# Autodesk Inventor assembly: asse_s_tstage
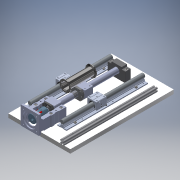
[picture p0: Inventor's stored thumbnail of the model, 180x180]
Saved by Autodesk Inventor 2019 (Build 230136000, 136)
## iProperties
Created: 2022-09-02
Part Number: asse_s_tstage
Document SubType Name: Assembly
Designer: kananovicha
Author: kananovicha
## Documents named in this file (10)
- C:\Users\kananovicha\Documents\work\workAppState\prj_shocksL\s_tstage\drawingsGit\s_tstage\asse_s_tstage\asse_s_tstage.iam
- C:\Users\kananovicha\Documents\work\workAppState\prj_shocksL\s_tstage\drawingsGit\s_tstage\mplate\mplate.ipt
- C:\Users\kananovicha\Documents\work\workAppState\prj_shocksL\s_tstage\drawingsGit\s_tstage\3rdParty\ballScrewAssembly\2510 L=400.iam
- C:\Users\kananovicha\Documents\work\workAppState\prj_shocksL\s_tstage\drawingsGit\s_tstage\allmainparams\allmainparams.ipt
- C:\Users\kananovicha\Documents\work\workAppState\prj_shocksL\s_tstage\drawingsGit\s_tstage\3rdParty\KF40nipple\qf40-150-n.iam
- C:\Users\kananovicha\Documents\work\workAppState\prj_shocksL\s_tstage\drawingsGit\s_tstage\3rdParty\br20-shaft-and-support-rail-resizable-1.snapshot.13\BR20\BR20-400.iam
- C:\Users\kananovicha\Documents\work\workAppState\prj_shocksL\s_tstage\drawingsGit\s_tstage\3rdParty\mod-sbr20uu-open-linear-bearing-1.snapshot.2\SBR20UU.iam
- C:\Users\kananovicha\Documents\work\workAppState\prj_shocksL\s_tstage\drawingsGit\s_tstage\tslot2020short\tslot2020short.ipt
- C:\Users\kananovicha\Documents\work\workAppState\prj_shocksL\s_tstage\drawingsGit\s_tstage\3rdParty\fasteners\ANSI B18.3.1M - M8x1.25 x 50(1).ipt
- C:\Users\kananovicha\Documents\work\workAppState\prj_shocksL\s_tstage\drawingsGit\s_tstage\3rdParty\fasteners\91290A328_Alloy Steel Socket Head Screw.ipt
## Components (26 placed, 8 different names)
1. mplate:1 — Flush:1, Mate:1, Mate:2, Mate:3, Mate:4, Angle:1, Angle:2, Angle:3, Flush:4, Mate:7, Flush:5, Flush:6
2. 2510 L=400:1 [sub-assembly] — Flush:1, Mate:1, Mate:2, Mate:5, Mate:6, Insert:1, Insert:2, Insert:3, Insert:4, Insert:5, Insert:6
3. qf40-150-n:1 [sub-assembly]
4. BR20-400:1 [sub-assembly] — Mate:3, Cylindrical:1, Angle:2, Mate:5, Mate:8, Flush:5, Insert:7
5. BR20-400:2 [sub-assembly] — Mate:4, Cylindrical:2, Mate:6, Flush:6, Insert:8
6. SBR20UU:1 [sub-assembly] — Cylindrical:1, Angle:1
7. SBR20UU:2 [sub-assembly] — Cylindrical:2, Angle:3
8. tslot2020short:1 — Flush:4, Mate:7, Mate:8
9. ANSI B18.3.1M - M8x1.25 x 50(1):1 — Insert:1
10. ANSI B18.3.1M - M8x1.25 x 50(1):2 — Insert:2
11. ANSI B18.3.1M - M8x1.25 x 50(1):3 — Insert:3
12. ANSI B18.3.1M - M8x1.25 x 50(1):4 — Insert:4
13. ANSI B18.3.1M - M8x1.25 x 50(1):5 — Insert:5
14. ANSI B18.3.1M - M8x1.25 x 50(1):6 — Insert:6
15. 91290A328_Alloy Steel Socket Head Screw:1 — Insert:7
16. 91290A328_Alloy Steel Socket Head Screw:3
17. 91290A328_Alloy Steel Socket Head Screw:4
18. 91290A328_Alloy Steel Socket Head Screw:5
19. 91290A328_Alloy Steel Socket Head Screw:6
20. 91290A328_Alloy Steel Socket Head Screw:7
21. 91290A328_Alloy Steel Socket Head Screw:2 — Insert:8
22. 91290A328_Alloy Steel Socket Head Screw:8
23. 91290A328_Alloy Steel Socket Head Screw:9
24. 91290A328_Alloy Steel Socket Head Screw:10
25. 91290A328_Alloy Steel Socket Head Screw:11
26. 91290A328_Alloy Steel Socket Head Screw:12
## Component patterns: (6 elements, first: 91290A328_Alloy Steel Socket Head Screw:1), (6 elements, first: 91290A328_Alloy Steel Socket Head Screw:2)
## Relationships (25: Mate 8, Insert 8, Flush 4, Angle 3, CylindricalJoint 2)
- Flush:1 (68.58 mm): mplate:1 ↔ 2510 L=400:1
- Mate:1: mplate:1 ↔ 2510 L=400:1
- Mate:2: mplate:1 ↔ 2510 L=400:1
- Mate:3: mplate:1 ↔ BR20-400:1
- Mate:4: mplate:1 ↔ BR20-400:2
- Cylindrical:1: BR20-400:1 ↔ SBR20UU:1
- Angle:1 (0 deg): mplate:1 ↔ SBR20UU:1
- Angle:2 (0 deg): mplate:1 ↔ BR20-400:1
- Cylindrical:2: BR20-400:2 ↔ SBR20UU:2
- Angle:3 (0 deg): mplate:1 ↔ SBR20UU:2
- Mate:5 (12.7 mm): 2510 L=400:1 ↔ BR20-400:1
- Mate:6 (12.7 mm): 2510 L=400:1 ↔ BR20-400:2
- Flush:4: mplate:1 ↔ tslot2020short:1
- Mate:7: mplate:1 ↔ tslot2020short:1
- Mate:8 (38.354 mm): BR20-400:1 ↔ tslot2020short:1
- Insert:1: 2510 L=400:1 ↔ ANSI B18.3.1M - M8x1.25 x 50(1):1
- Insert:2: 2510 L=400:1 ↔ ANSI B18.3.1M - M8x1.25 x 50(1):2
- Insert:3: 2510 L=400:1 ↔ ANSI B18.3.1M - M8x1.25 x 50(1):3
- Insert:4: 2510 L=400:1 ↔ ANSI B18.3.1M - M8x1.25 x 50(1):4
- Insert:5: 2510 L=400:1 ↔ ANSI B18.3.1M - M8x1.25 x 50(1):5
- Insert:6: 2510 L=400:1 ↔ ANSI B18.3.1M - M8x1.25 x 50(1):6
- Flush:5 (68.25 mm): mplate:1 ↔ BR20-400:1
- Flush:6 (68.25 mm): mplate:1 ↔ BR20-400:2
- Insert:7: BR20-400:1 ↔ 91290A328_Alloy Steel Socket Head Screw:1
- Insert:8: BR20-400:2 ↔ 91290A328_Alloy Steel Socket Head Screw:2
## Named parameters: asse_sfu_offset_wid = 68.58 mm, asse_sbr_railSeparation = 12.7 mm, asse_tslo_separation = 38.354 mm, asse_brm_l_offset = 68.25 mm, brm_hole_v_offset = 50 mm, brm_hole_h_offset = 7.493 mm, brm_hole_h_spacing = 29.9974 mm, brm_hole_v_spacing = 150 mm
